# Autodesk Inventor assembly: Сборка2
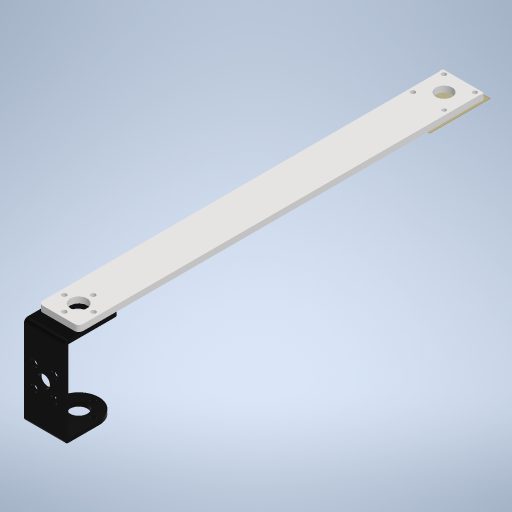
[picture p0: Inventor's stored thumbnail of the model, 512x512]
Saved by Autodesk Inventor 2023 (Build 270158000, 158)
## iProperties
Created: 2025-02-02
Part Number: Сборка2
Document SubType Name: Assembly
Designer: baranovaem
Author: baranovaem
## Documents named in this file (3)
- \\sch239.net\UserHomes\Students\other\baranovaem\cheburashka\Cheburashka-main\Cheburashka_construction\korpus\Сборка2.iam
- \\sch239.net\UserHomes\Students\other\baranovaem\cheburashka\Cheburashka-main\Cheburashka_construction\korpus\acc1.ipt
- \\sch239.net\UserHomes\Students\other\baranovaem\cheburashka\Cheburashka-main\Cheburashka_construction\korpus\резать и печатать\рука.ipt
## Components (2 placed, 2 different names)
1. acc1:1 — Совмещение:1, Угол:1
2. рука:1 — Заподлицо:1, Заподлицо:2
## Relationships (4: Flush 2, Mate 1, Angle 1)
- Совмещение:1 [Mate]: acc1:1
- Угол:1 [Angle] (0 deg): acc1:1
- Заподлицо:1 [Flush]: рука:1
- Заподлицо:2 [Flush]: рука:1
